# Autodesk Inventor assembly: FingerProto1
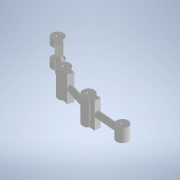
[picture p0: Inventor's stored thumbnail of the model, 180x180]
Saved by Autodesk Inventor 2021 (Build 250183000, 183)
## iProperties
Created: 2022-08-29
Part Number: FingerProto1
Document SubType Name: Assembly
Designer: alyn649
Author: alyn649
## Documents named in this file (2)
- \\files.auckland.ac.nz\myhome\Documents\GitHub\hand\FingerProto1.iam
- \\files.auckland.ac.nz\myhome\Documents\GitHub\hand\Phalalnge_28mm.ipt
## Components (3 placed, 1 different names)
1. Phalalnge_28mm:1 — Rotational:1
2. Phalalnge_28mm:2 — Rotational:2
3. Phalalnge_28mm:3 — Rotational:1, Rotational:2
## Relationships (2: RevoluteJoint 2)
- Rotational:1 [RevoluteJoint]: Phalalnge_28mm:1 ↔ Phalalnge_28mm:3
- Rotational:2 [RevoluteJoint]: Phalalnge_28mm:2 ↔ Phalalnge_28mm:3
